# Autodesk Inventor assembly: assembly
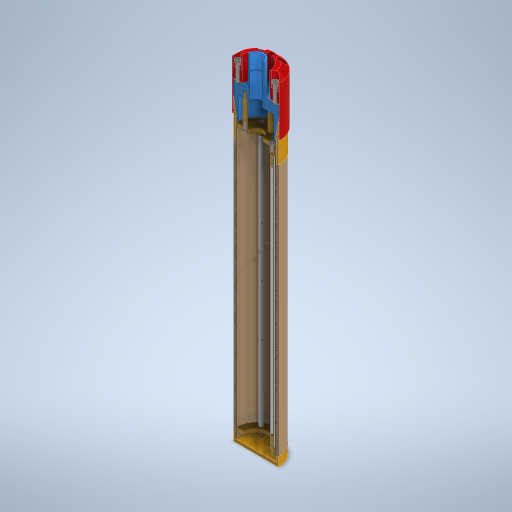
[picture p0: Inventor's stored thumbnail of the model, 512x512]
Saved by Autodesk Inventor 2024 (Build 280153000, 153)
## iProperties
Created: 2023-09-22
Part Number: assembly
Document SubType Name: Assembly
Designer: schanen
Author: schanen
## Documents named in this file (8)
- C:\Users\schanen\Documents\Inventor\he4inserts\assembly.iam
- C:\Users\schanen\Documents\Inventor\he4inserts\Clamp.ipt
- C:\Users\schanen\Documents\Inventor\he4inserts\Screw_StainlessSteal_M4_SocketCap_20mm.ipt
- C:\Users\schanen\Documents\Inventor\he4inserts\FlangeCone.ipt
- C:\Users\schanen\Documents\Inventor\he4inserts\BodyCylinder.ipt
- C:\Users\schanen\Documents\Inventor\he4inserts\CapCone.ipt
- C:\Users\schanen\Documents\Inventor\he4inserts\CapCenter.ipt
- C:\Users\schanen\Documents\Inventor\he4inserts\insertAssembly-2.iam
## Components (13 placed, 7 different names)
1. Clamp:1 — Mate:1, Mate:3, Mate:4, Flush:1, Mate:5, Angle:1, Mate:17
2. Clamp:2 — Mate:3, Mate:4, Flush:1
3. FlangeCone:1 — Mate:5, Mate:6, Mate:7, Mate:17, Mate:18, Mate:24, Mate:25, Mate:26
4. CapCone:1 — Mate:18, Mate:19, Mate:21, Mate:22
5. CapCenter:1 — Mate:22, Mate:23
6. BodyCylinder:1 — Mate:19, Mate:21, Mate:23
7. insertAssembly-2:1 [sub-assembly] — Mate:24, Mate:25, Mate:26
8. Screw_StainlessSteal_M4_SocketCap_20mm:1 — Mate:1, Mate:6
9. Screw_StainlessSteal_M4_SocketCap_20mm:2
10. Screw_StainlessSteal_M4_SocketCap_20mm:3
11. Screw_StainlessSteal_M4_SocketCap_20mm:4
12. Screw_StainlessSteal_M4_SocketCap_20mm:5
13. Screw_StainlessSteal_M4_SocketCap_20mm:6
## Component patterns: (6 elements, first: Screw_StainlessSteal_M4_SocketCap_20mm:1)
## Relationships (17: Mate 15, Flush 1, Angle 1)
- Mate:1: Clamp:1 ↔ Screw_StainlessSteal_M4_SocketCap_20mm:1
- Mate:3: Clamp:1 ↔ Clamp:2
- Mate:4 (5 mm): Clamp:1 ↔ Clamp:2
- Flush:1: Clamp:1 ↔ Clamp:2
- Mate:5: Clamp:1 ↔ FlangeCone:1
- Mate:6: FlangeCone:1 ↔ Screw_StainlessSteal_M4_SocketCap_20mm:1
- Mate:7: FlangeCone:1
- Angle:1 (0 deg): Clamp:1
- Mate:17: Clamp:1 ↔ FlangeCone:1
- Mate:18: FlangeCone:1 ↔ CapCone:1
- Mate:19: CapCone:1 ↔ BodyCylinder:1
- Mate:21: CapCone:1 ↔ BodyCylinder:1
- Mate:22: CapCone:1 ↔ CapCenter:1
- Mate:23: CapCenter:1 ↔ BodyCylinder:1
- Mate:24: FlangeCone:1 ↔ insertAssembly-2:1
- Mate:25: FlangeCone:1 ↔ insertAssembly-2:1
- Mate:26: FlangeCone:1 ↔ insertAssembly-2:1
